# Autodesk Inventor assembly: Pancake_Timing Assy_Lever Shaft 2_3 Lanes
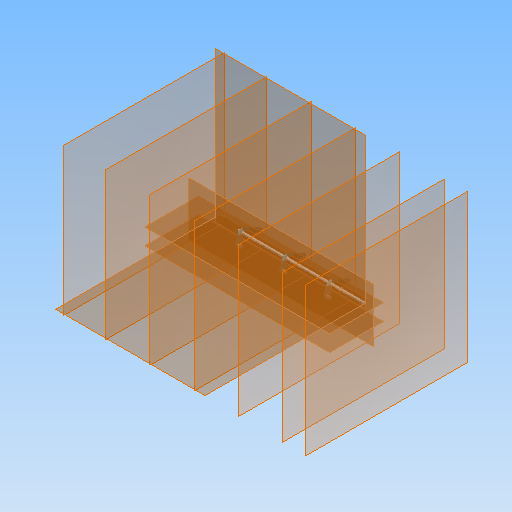
[picture p0: Inventor's stored thumbnail of the model, 512x512]
Saved by Autodesk Inventor 2018.1 (Build 221171000, 171)
## iProperties
Created: 2019-02-11
Part Number: Pancake_Timing Assy_Lever Shaft 2_3 Lanes
Document SubType Name: Assembly
Designer: James
Author: James
## Documents named in this file (7)
- C:\Users\admin\Desktop\Ball Sorting Machine\Ball-Sorting-Machine\Pancake Sort\Pancake - 3 Lanes\Pancake_Timing Assy_Lever Shaft 2_3 Lanes.iam
- C:\Users\admin\Desktop\Ball Sorting Machine\Ball-Sorting-Machine\Pancake Sort\BS 3673 - 6mm External Circlip.ipt
- C:\Users\admin\Desktop\Ball Sorting Machine\Ball-Sorting-Machine\Timing Gate\M3 x 0.5mm Zinc Plated Steel Washer.ipt
- C:\Users\admin\Desktop\Ball Sorting Machine\Ball-Sorting-Machine\Timing Gate\Socket Button Head - (A2) - M3 x 10.ipt
- C:\Users\admin\Desktop\Ball Sorting Machine\Ball-Sorting-Machine\Timing Gate\Timing_Lever Weight.ipt
- C:\Users\admin\Desktop\Ball Sorting Machine\Ball-Sorting-Machine\Pancake Sort\Pancake_Lever.ipt
- C:\Users\admin\Desktop\Ball Sorting Machine\Ball-Sorting-Machine\Pancake Sort\Pancake - 3 Lanes\Pancake_Lever Shaft 2_3 Lanes.ipt
## Components (21 placed, 6 different names)
1. Pancake_Lever Shaft 2_3 Lanes:1 — Mate:45, Flush:18, Mate:46, Mate:47, Mate:48, Mate:49, Mate:52, Mate:53, Mate:54, Mate:55
2. BS 3673 - 6mm External Circlip:11 — Mate:52, Mate:55, Flush:20
3. BS 3673 - 6mm External Circlip:12 — Mate:53, Mate:54, Flush:20
4. BS 3673 - 6mm External Circlip:1 — Flush:10, Mate:46, Mate:49, Flush:19, Angle:3
5. Pancake_Lever:1 — Mate:13, Mate:14, Mate:16, Mate:45, Flush:18, Mate:51
6. BS 3673 - 6mm External Circlip:2 — Flush:10, Angle:2, Mate:47, Mate:48, Flush:19
7. Socket Button Head - (A2) - M3 x 10:1 — Mate:15, Mate:16, Mate:50
8. M3 x 0.5mm Zinc Plated Steel Washer:1 — Mate:13, Mate:14, Mate:15
9. Timing_Lever Weight:1 — Mate:50, Mate:51
10. BS 3673 - 6mm External Circlip:3
11. Pancake_Lever:2
12. BS 3673 - 6mm External Circlip:4
13. Socket Button Head - (A2) - M3 x 10:2
14. M3 x 0.5mm Zinc Plated Steel Washer:2
15. Timing_Lever Weight:2
16. BS 3673 - 6mm External Circlip:5
17. Pancake_Lever:3
18. BS 3673 - 6mm External Circlip:6
19. Socket Button Head - (A2) - M3 x 10:3
20. M3 x 0.5mm Zinc Plated Steel Washer:3
21. Timing_Lever Weight:3
## Component patterns: (3 elements, first: BS 3673 - 6mm External Circlip:1 + Pancake_Lever:1 + BS 3673 - 6mm External Circlip:2 + Socket Button Head - (A2) - M3 x 10:1 + M3 x 0.5mm Zinc Plated Steel Washer:1 + Timing_Lever Weight:1)
## Relationships (27: Mate 15, Flush 10, Angle 2)
- [Flush]: Pancake_Lever Shaft 2_3 Lanes:1
- Flush:10: BS 3673 - 6mm External Circlip:1 ↔ BS 3673 - 6mm External Circlip:2
- Angle:2 (180 deg): BS 3673 - 6mm External Circlip:2
- Mate:13: Pancake_Lever:1 ↔ M3 x 0.5mm Zinc Plated Steel Washer:1
- Mate:14: Pancake_Lever:1 ↔ M3 x 0.5mm Zinc Plated Steel Washer:1
- Mate:15: Socket Button Head - (A2) - M3 x 10:1 ↔ M3 x 0.5mm Zinc Plated Steel Washer:1
- Mate:16: Pancake_Lever:1 ↔ Socket Button Head - (A2) - M3 x 10:1
- Flush:11 (-58 mm)
- Flush:12 (-5 mm)
- Flush:13 (30 mm)
- [Flush]: Pancake_Lever Shaft 2_3 Lanes:1
- [Flush]: Pancake_Lever Shaft 2_3 Lanes:1
- Mate:45: Pancake_Lever Shaft 2_3 Lanes:1 ↔ Pancake_Lever:1
- Flush:18: Pancake_Lever Shaft 2_3 Lanes:1 ↔ Pancake_Lever:1
- Mate:46: Pancake_Lever Shaft 2_3 Lanes:1 ↔ BS 3673 - 6mm External Circlip:1
- Mate:47: Pancake_Lever Shaft 2_3 Lanes:1 ↔ BS 3673 - 6mm External Circlip:2
- Mate:48: Pancake_Lever Shaft 2_3 Lanes:1 ↔ BS 3673 - 6mm External Circlip:2
- Mate:49: Pancake_Lever Shaft 2_3 Lanes:1 ↔ BS 3673 - 6mm External Circlip:1
- Flush:19: BS 3673 - 6mm External Circlip:1 ↔ BS 3673 - 6mm External Circlip:2
- Angle:3 (0 deg): BS 3673 - 6mm External Circlip:1
- Mate:50: Socket Button Head - (A2) - M3 x 10:1 ↔ Timing_Lever Weight:1
- Mate:51: Pancake_Lever:1 ↔ Timing_Lever Weight:1
- Mate:52: Pancake_Lever Shaft 2_3 Lanes:1 ↔ BS 3673 - 6mm External Circlip:11
- Mate:53: Pancake_Lever Shaft 2_3 Lanes:1 ↔ BS 3673 - 6mm External Circlip:12
- Mate:54: Pancake_Lever Shaft 2_3 Lanes:1 ↔ BS 3673 - 6mm External Circlip:12
- Mate:55: Pancake_Lever Shaft 2_3 Lanes:1 ↔ BS 3673 - 6mm External Circlip:11
- Flush:20: BS 3673 - 6mm External Circlip:11 ↔ BS 3673 - 6mm External Circlip:12
